# Autodesk Inventor assembly: TL20240701-10100AT-000
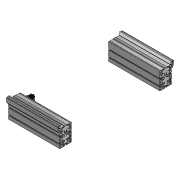
[picture p0: Inventor's stored thumbnail of the model, 180x180]
Saved by Autodesk Inventor 2022.5 (Build 265521000, 521)
## iProperties
Category: CONVEYOR ASSY
Company: 현대트랜시스(대유)
RuleStatus: InUse
Created: 2024-07-26
Part Number: TL20240701-10100AT-000
Project: SW-PJT
Checked By: 김형민
Engr Approved By: 김시현
User Status: 1 x78
Material: SS400
Description: 5
Document SubType Name: Assembly
Mfg Approved By: 호상태
Designer: USER106
Stock Number: 000
Mass: 455.999 g
Surface Area: 237.231 cm^2
Volume: 78.1044 cm^3
Density: 5.83832 g/cm^3
Deteil Description: Detail Description
Detail Description: Assembly products
Title: ANTI BACK ASSY
Subject: SW차종 시트조립라인
Author: USER106
Revision Number: A
## Documents named in this file (9)
- D:\V\Designs\프로젝트 자산\자동화 & 스마트팩토리\현대트랜시스(구 다이모스, 파워텍)\현대트랜시스(대유화성공장)_SW 시트조립라인\2.제작도면\1. 1ST LINE\ANTI BACK\TL20240701-10100AT\TL20240701-10100AT-000.iam
- D:\V\Designs\프로젝트 자산\자동화 & 스마트팩토리\현대트랜시스(구 다이모스, 파워텍)\현대트랜시스(대유화성공장)_SW 시트조립라인\2.제작도면\1. 1ST LINE\ANTI BACK\TL20240701-10100AT\TL20240701-10100AT-001.ipt
- D:\V\Designs\프로젝트 자산\자동화 & 스마트팩토리\현대트랜시스(구 다이모스, 파워텍)\현대트랜시스(대유화성공장)_SW 시트조립라인\2.제작도면\1. 1ST LINE\ANTI BACK\TL20240701-10100AT\TL20240701-10100AT-002.ipt
- D:\V\Designs\프로젝트 자산\자동화 & 스마트팩토리\현대트랜시스(구 다이모스, 파워텍)\현대트랜시스(대유화성공장)_SW 시트조립라인\2.제작도면\1. 1ST LINE\ANTI BACK\TL20240701-10100AT\TL20240701-10100AT-003.ipt
- D:\V\Designs\프로젝트 자산\자동화 & 스마트팩토리\현대트랜시스(구 다이모스, 파워텍)\현대트랜시스(대유화성공장)_SW 시트조립라인\2.제작도면\기타(도면용 구성품)\PROFILE_Simplify-A.ipt
- D:\V\Designs\구매품(업체별)\LUBO\DU BUSH_MB0808-15FDU_LUBO.ipt
- D:\V\Content Center Files\en-US\KS B 1320  A\KS B 1320 - A 3 x  16.ipt
- D:\V\Content Center Files\en-US\KS B 1012  C\KS B 1012 - C M8C.ipt
- D:\V\Content Center Files\en-US\KS B 1003\KS B 1003 - M 8 x 35.ipt
## Components (9 placed, 8 different names)
1. DU BUSH_MB0808-15FDU_LUBO:1 — Mate:10, Mate:11
2. DU BUSH_MB0808-15FDU_LUBO:3 — Mate:12, Mate:13
3. KS B 1003 - Metric M 8 x 35:1 — Mate:5, Flush:5, Mate:6
4. KS B 1012 C - Metric C M8:1 — Mate:6, Mate:7
5. KS B 1320 A A 3 x  16:1 — Mate:14, Flush:7
6. PROFILE_Simplify-A:1 — Mate:8, Flush:6, Mate:9
7. TL20240701-10100AT-001.ipt:1 — Flush:1, Flush:2, Flush:3, Mate:1, Flush:4, Mate:3, Angle:1, Mate:4, Mate:8, Flush:6, Mate:9, Mate:11, Mate:13, Mate:14, Flush:7, Mate:15
8. TL20240701-10100AT-002.ipt:1 — Mate:1, Flush:4, Mate:2, Mate:10, Mate:12
9. TL20240701-10100AT-003.ipt:1 — Mate:2, Mate:3, Angle:1, Mate:4, Mate:5, Flush:5, Mate:7, Mate:15
## Relationships (23: Mate 15, Flush 7, Angle 1)
- Flush:1: TL20240701-10100AT-001.ipt:1
- Flush:2: TL20240701-10100AT-001.ipt:1
- Flush:3: TL20240701-10100AT-001.ipt:1
- Mate:1: TL20240701-10100AT-001.ipt:1 ↔ TL20240701-10100AT-002.ipt:1
- Flush:4: TL20240701-10100AT-001.ipt:1 ↔ TL20240701-10100AT-002.ipt:1
- Mate:2: TL20240701-10100AT-002.ipt:1 ↔ TL20240701-10100AT-003.ipt:1
- Mate:3 (1 mm): TL20240701-10100AT-001.ipt:1 ↔ TL20240701-10100AT-003.ipt:1
- Angle:1 (0 deg): TL20240701-10100AT-001.ipt:1 ↔ TL20240701-10100AT-003.ipt:1
- Mate:4: TL20240701-10100AT-001.ipt:1 ↔ TL20240701-10100AT-003.ipt:1
- Mate:5: KS B 1003 - Metric M 8 x 35:1 ↔ TL20240701-10100AT-003.ipt:1
- Flush:5: KS B 1003 - Metric M 8 x 35:1 ↔ TL20240701-10100AT-003.ipt:1
- Mate:6: KS B 1003 - Metric M 8 x 35:1 ↔ KS B 1012 C - Metric C M8:1
- Mate:7: KS B 1012 C - Metric C M8:1 ↔ TL20240701-10100AT-003.ipt:1
- Mate:8: PROFILE_Simplify-A:1 ↔ TL20240701-10100AT-001.ipt:1
- Flush:6: PROFILE_Simplify-A:1 ↔ TL20240701-10100AT-001.ipt:1
- Mate:9: PROFILE_Simplify-A:1 ↔ TL20240701-10100AT-001.ipt:1
- Mate:10: DU BUSH_MB0808-15FDU_LUBO:1 ↔ TL20240701-10100AT-002.ipt:1
- Mate:11: DU BUSH_MB0808-15FDU_LUBO:1 ↔ TL20240701-10100AT-001.ipt:1
- Mate:12: DU BUSH_MB0808-15FDU_LUBO:3 ↔ TL20240701-10100AT-002.ipt:1
- Mate:13: DU BUSH_MB0808-15FDU_LUBO:3 ↔ TL20240701-10100AT-001.ipt:1
- Mate:14: KS B 1320 A A 3 x  16:1 ↔ TL20240701-10100AT-001.ipt:1
- Flush:7: KS B 1320 A A 3 x  16:1 ↔ TL20240701-10100AT-001.ipt:1
- Mate:15: TL20240701-10100AT-001.ipt:1 ↔ TL20240701-10100AT-003.ipt:1
